# Autodesk Inventor assembly: Battery holder
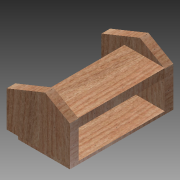
[picture p0: Inventor's stored thumbnail of the model, 180x180]
Saved by Autodesk Inventor 2014 (Build 180170000, 170)
## iProperties
Created: 2016-02-01
Part Number: Battery holder
Document SubType Name: Assembly
Designer: sametj
Author: sametj
## Documents named in this file (4)
- Z:\Robot\Battery holder.iam
- Z:\Robot\side battery.ipt
- Z:\Robot\inside battery holder.ipt
- Z:\Robot\bottom2 battery holder.ipt
## Components (4 placed, 3 different names)
1. side battery:1 — Flush:1, Flush:2, Mate:1, Flush:3, Mate:2, Flush:6
2. side battery:2 — Flush:1, Flush:2, Flush:4, Flush:5
3. inside battery holder:1 — Mate:2, Mate:3, Flush:6
4. bottom2 battery holder:1 — Mate:1, Flush:3, Flush:4, Flush:5, Mate:3
## Relationships (9: Flush 6, Mate 3)
- Flush:1: side battery:1 ↔ side battery:2
- Flush:2: side battery:1 ↔ side battery:2
- Mate:1: side battery:1 ↔ bottom2 battery holder:1
- Flush:3: side battery:1 ↔ bottom2 battery holder:1
- Flush:4: side battery:2 ↔ bottom2 battery holder:1
- Flush:5: side battery:2 ↔ bottom2 battery holder:1
- Mate:2: side battery:1 ↔ inside battery holder:1
- Mate:3 (63.5 mm): inside battery holder:1 ↔ bottom2 battery holder:1
- Flush:6: side battery:1 ↔ inside battery holder:1
